# Autodesk Inventor assembly: Comparisson
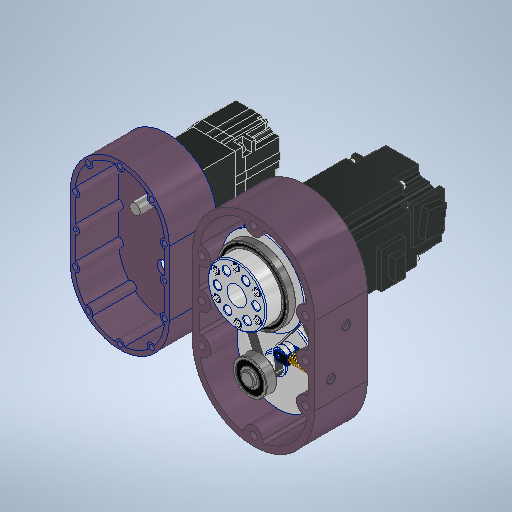
[picture p0: Inventor's stored thumbnail of the model, 512x512]
Saved by Autodesk Inventor 2026 (Build 300175000, 175)
## iProperties
Created: 2025-12-03
Part Number: Comparisson
Document SubType Name: Assembly
Designer: DanielFGarzon
Author: DanielFGarzon
## Documents named in this file (4)
- D:\POLIMI\3RD SEMESTER\Industrial Robotics\Project\Mine\Comparisson.iam
- D:\POLIMI\3RD SEMESTER\Industrial Robotics\Project\Mine\Reducer_02\01_Housing.ipt
- D:\POLIMI\3RD SEMESTER\Industrial Robotics\Project\Mine\Reducer.iam
- D:\POLIMI\3RD SEMESTER\Industrial Robotics\Project\Mine\Robot_Desing\Motors_Info\04_HG-KR053\04_HG-KR053\04_HG-KR053.ipt
## Components (3 placed, 3 different names)
1. 01_Housing:1 — Mate:1, Flush:1, Mate:2, Mate:3, Mate:4
2. Reducer:1 [sub-assembly] — Mate:1, Flush:1
3. 04_HG-KR053:1 — Mate:2, Mate:3, Mate:4
## Relationships (5: Mate 4, Flush 1)
- Mate:1 (22 mm): 01_Housing:1 ↔ Reducer:1
- Flush:1: 01_Housing:1 ↔ Reducer:1
- Mate:2: 01_Housing:1 ↔ 04_HG-KR053:1
- Mate:3: 01_Housing:1 ↔ 04_HG-KR053:1
- Mate:4: 01_Housing:1 ↔ 04_HG-KR053:1
